# Autodesk Inventor assembly: Full_Design
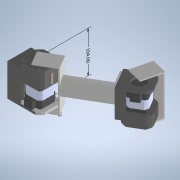
[picture p0: Inventor's stored thumbnail of the model, 180x180]
Saved by Autodesk Inventor 2022 (Build 260153000, 153)
## iProperties
Created: 2022-02-10
Part Number: Full_Design
Document SubType Name: Assembly
Designer: Mlees
Author: Mlees
## Documents named in this file (11)
- C:\Users\Mlees\Desktop\504Engineering\Stepper-Servo_Based_Robotic_Arm\Designs\Version_5\Full_Design.iam
- C:\Users\Mlees\Desktop\504Engineering\Stepper-Servo_Based_Robotic_Arm\Designs\Version_5\Downloaded_Parts\124125202-9-stp-mtr-17040w\stp-mtr-17040w.ipt
- C:\Users\Mlees\Desktop\504Engineering\Stepper-Servo_Based_Robotic_Arm\Designs\Version_5\Created_Parts\24_Teeth_Sun_Gear.ipt
- C:\Users\Mlees\Desktop\504Engineering\Stepper-Servo_Based_Robotic_Arm\Designs\Version_5\Created_Parts\36_Teeth_Planet_Gear.ipt
- C:\Users\Mlees\Desktop\504Engineering\Stepper-Servo_Based_Robotic_Arm\Designs\Version_5\Created_Parts\Gear_Cover_modified.ipt
- C:\Users\Mlees\Desktop\504Engineering\Stepper-Servo_Based_Robotic_Arm\Designs\Version_5\Created_Parts\Plamet_Carrier.ipt
- C:\Users\Mlees\Desktop\504Engineering\Stepper-Servo_Based_Robotic_Arm\Designs\Version_5\Created_Parts\Planet_Carrier_Modifed_with_sun_gear.ipt
- C:\Users\Mlees\Desktop\504Engineering\Stepper-Servo_Based_Robotic_Arm\Designs\Version_5\Created_Parts\Combined_Gear_Box.ipt
- C:\Users\Mlees\Desktop\504Engineering\Stepper-Servo_Based_Robotic_Arm\Designs\Version_5\Created_Parts\Tilt_Bracket_Output.ipt
- C:\Users\Mlees\Desktop\504Engineering\Stepper-Servo_Based_Robotic_Arm\Designs\Version_5\Created_Parts\96Gears_Stage_1_modified_Joint_2.ipt
- C:\Users\Mlees\Desktop\504Engineering\Stepper-Servo_Based_Robotic_Arm\Designs\Version_5\Created_Parts\Tilt_Bracket_Output_2.ipt
## Components (22 placed, 10 different names)
1. stp-mtr-17040w:1 — Rigid:2, Rigid:5, Rotational:1
2. 24_Teeth_Sun_Gear:1 — Rigid:2
3. 36_Teeth_Planet_Gear:1 — Rigid:14
4. Gear_Cover_modified:1
5. Plamet_Carrier:1 — Rigid:7, Rigid:12, Rigid:13, Rigid:14, Rotational:2
6. Planet_Carrier_Modifed_with_sun_gear:1 — Rigid:5, Rigid:7, Rigid:9, Rigid:10, Rigid:11
7. 36_Teeth_Planet_Gear:2 — Rigid:13
8. 36_Teeth_Planet_Gear:3 — Rigid:12
9. 36_Teeth_Planet_Gear:4 — Rigid:9
10. 36_Teeth_Planet_Gear:5 — Rigid:10
11. 36_Teeth_Planet_Gear:6 — Rigid:11
12. Combined_Gear_Box:1 — Rotational:1
13. Tilt_Bracket_Output:1 — Rigid:15, Rotational:2
14. 96Gears_Stage_1_modified_Joint_2:1 — Rigid:15, Rigid:16, Rigid:17
15. stp-mtr-17040w:2 — Rigid:16, Rotational:3
16. 24_Teeth_Sun_Gear:2 — Rotational:3, Rotational:7
17. 36_Teeth_Planet_Gear:7 — Rotational:6
18. Gear_Cover_modified:2 — Rigid:17
19. Plamet_Carrier:2 — Rotational:4, Rotational:5, Rotational:6, Rotational:7, Rotational:8
20. 36_Teeth_Planet_Gear:8 — Rotational:4
21. 36_Teeth_Planet_Gear:9 — Rotational:5
22. Tilt_Bracket_Output_2:1 — Rotational:8
## Relationships (20: WeldJoint 12, RevoluteJoint 8)
- Rigid:2 [WeldJoint]: stp-mtr-17040w:1 ↔ 24_Teeth_Sun_Gear:1
- Rigid:5 [WeldJoint]: stp-mtr-17040w:1 ↔ Planet_Carrier_Modifed_with_sun_gear:1
- Rigid:7 [WeldJoint]: Plamet_Carrier:1 ↔ Planet_Carrier_Modifed_with_sun_gear:1
- Rigid:9 [WeldJoint]: Planet_Carrier_Modifed_with_sun_gear:1 ↔ 36_Teeth_Planet_Gear:4
- Rigid:10 [WeldJoint]: Planet_Carrier_Modifed_with_sun_gear:1 ↔ 36_Teeth_Planet_Gear:5
- Rigid:11 [WeldJoint]: Planet_Carrier_Modifed_with_sun_gear:1 ↔ 36_Teeth_Planet_Gear:6
- Rigid:12 [WeldJoint]: Plamet_Carrier:1 ↔ 36_Teeth_Planet_Gear:3
- Rigid:13 [WeldJoint]: Plamet_Carrier:1 ↔ 36_Teeth_Planet_Gear:2
- Rigid:14 [WeldJoint]: 36_Teeth_Planet_Gear:1 ↔ Plamet_Carrier:1
- Rotational:1 [RevoluteJoint]: stp-mtr-17040w:1 ↔ Combined_Gear_Box:1
- Rigid:15 [WeldJoint]: Tilt_Bracket_Output:1 ↔ 96Gears_Stage_1_modified_Joint_2:1
- Rotational:2 [RevoluteJoint]: Plamet_Carrier:1 ↔ Tilt_Bracket_Output:1
- Rigid:16 [WeldJoint]: 96Gears_Stage_1_modified_Joint_2:1 ↔ stp-mtr-17040w:2
- Rotational:3 [RevoluteJoint]: stp-mtr-17040w:2 ↔ 24_Teeth_Sun_Gear:2
- Rotational:4 [RevoluteJoint]: Plamet_Carrier:2 ↔ 36_Teeth_Planet_Gear:8
- Rotational:5 [RevoluteJoint]: Plamet_Carrier:2 ↔ 36_Teeth_Planet_Gear:9
- Rotational:6 [RevoluteJoint]: 36_Teeth_Planet_Gear:7 ↔ Plamet_Carrier:2
- Rotational:7 [RevoluteJoint]: 24_Teeth_Sun_Gear:2 ↔ Plamet_Carrier:2
- Rigid:17 [WeldJoint]: 96Gears_Stage_1_modified_Joint_2:1 ↔ Gear_Cover_modified:2
- Rotational:8 [RevoluteJoint]: Plamet_Carrier:2 ↔ Tilt_Bracket_Output_2:1
